# Autodesk Inventor assembly: WheelPod_ForDrawing
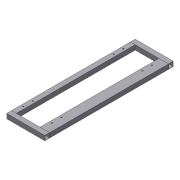
[picture p0: Inventor's stored thumbnail of the model, 180x180]
Saved by Autodesk Inventor 2012 (Build 160160000, 160)
## iProperties
Created: 2012-01-13
Part Number: WheelPod_ForDrawing
Document SubType Name: Assembly
Designer: JesseK
Author: JesseK
## Documents named in this file (4)
- Z:\UserData\Documents\Inventor\team1885frc\Robot2012\Conveyor2\WheelPod_ForDrawing.iam
- Z:\UserData\Documents\Inventor\team1885frc\Robot2012\DriveTrain\DriveTrain_SideRail.ipt
- Z:\UserData\Documents\Inventor\team1885frc\Robot2012\DriveTrain\Frame_SideRail_Inner_2x1.ipt
- Z:\UserData\Documents\Inventor\team1885frc\Robot2012\DriveTrain\FrontBumperRail.ipt
## Components (4 placed, 3 different names)
1. DriveTrain_SideRail:1 — Flush:3, Mate:2, Mate:3, Mate:4, Mate:5
2. Frame_SideRail_Inner_2x1:1 — Flush:1, Flush:2, Mate:1, Flush:4
3. FrontBumperRail:1 — Flush:1, Flush:2, Mate:1, Flush:3, Mate:2, Mate:3
4. FrontBumperRail:2 — Mate:4, Flush:4, Mate:5
## Relationships (9: Mate 5, Flush 4)
- Flush:1: Frame_SideRail_Inner_2x1:1 ↔ FrontBumperRail:1
- Flush:2: Frame_SideRail_Inner_2x1:1 ↔ FrontBumperRail:1
- Mate:1: Frame_SideRail_Inner_2x1:1 ↔ FrontBumperRail:1
- Flush:3: DriveTrain_SideRail:1 ↔ FrontBumperRail:1
- Mate:2: DriveTrain_SideRail:1 ↔ FrontBumperRail:1
- Mate:3: DriveTrain_SideRail:1 ↔ FrontBumperRail:1
- Mate:4: DriveTrain_SideRail:1 ↔ FrontBumperRail:2
- Flush:4: Frame_SideRail_Inner_2x1:1 ↔ FrontBumperRail:2
- Mate:5: DriveTrain_SideRail:1 ↔ FrontBumperRail:2
